# Autodesk Inventor assembly: 5A.00.03.01-IB-VTP-Rudder-Master-Assy
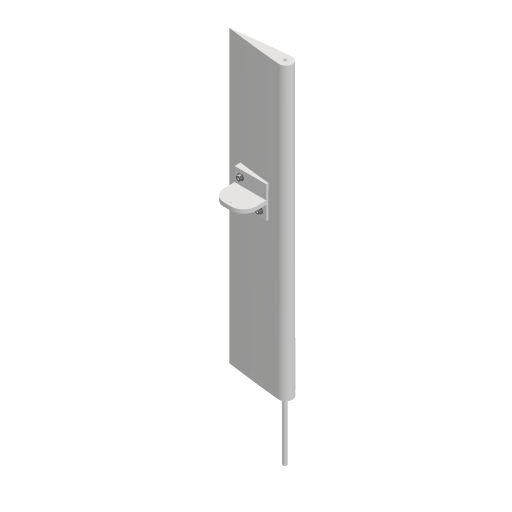
[picture p0: Inventor's stored thumbnail of the model, 512x512]
Saved by Autodesk Inventor 2024.3 (Build 283343000, 343)
## iProperties
Created: 2025-01-15
Part Number: 5A.00.03.01-IB-VTP-Rudder-Master-Assy
Document SubType Name: Assembly
Designer: inigo
Author: inigo
## Documents named in this file (11)
- C:\Users\inigo\OneDrive - University of Bristol\General - grp-Company A - AVDASI2 2024-25\CAD Files\Fuselage\VTP\5A.00.03.01-IB-VTP-Rudder-Master-Assy.iam
- C:\Users\inigo\OneDrive - University of Bristol\General - grp-Company A - AVDASI2 2024-25\CAD Files\Fuselage\VTP\5P.00.04.01-IB-VTP-Rudder-Right.ipt
- C:\Users\inigo\OneDrive - University of Bristol\General - grp-Company A - AVDASI2 2024-25\CAD Files\Fuselage\VTP\5P.00.05.01-IB-VTP-Rudder-Left.ipt
- C:\Users\inigo\OneDrive - University of Bristol\General - grp-Company A - AVDASI2 2024-25\CAD Files\Fuselage\VTP\5P.00.07.01-IB-VTP-Rudder-Bottom-Rib.ipt
- C:\Users\inigo\OneDrive - University of Bristol\General - grp-Company A - AVDASI2 2024-25\CAD Files\Fuselage\VTP\5P.00.08.01-IB-Rear-Spar.ipt
- C:\Users\inigo\OneDrive - University of Bristol\General - grp-Company A - AVDASI2 2024-25\CAD Files\Fuselage\VTP\5P.00.17.01-IB-VTP-Control-Horn.ipt
- C:\Users\inigo\OneDrive - University of Bristol\General - grp-Company A - AVDASI2 2024-25\CAD Files\Fuselage\VTP\5P.00.18.01-IB-VTP-Rudder-Top-Rib.ipt
- C:\Users\inigo\OneDrive - University of Bristol\General - grp-Company A - AVDASI2 2024-25\CAD Files\Fuselage\VTP\5P.00.21.01-IB-VTP-Rudder-Backplate.ipt
- C:\Users\inigo\Documents\Inventor\Content Center Files\R2024\en-US\ISO 4762(2)\ISO 4762 - M2 x 16ISO.ipt
- C:\Users\inigo\Documents\Inventor\Content Center Files\R2024\en-US\ISO 7089\ISO 7089 - 2 - 140 HV(1).ipt
- C:\Users\inigo\Documents\Inventor\Content Center Files\R2024\en-US\ISO 4032(2)\ISO 4032 - M2 - ISO.ipt
## Components (15 placed, 10 different names)
1. 5P.00.04.01-IB-VTP-Rudder-Right:1 — Mate:4, Mate:5, Flush:1, Mate:8, Mate:9, Mate:10, Mate:11, Mate:12, Flush:3
2. 5P.00.05.01-IB-VTP-Rudder-Left:1 — Mate:1, Mate:3, Mate:5, Flush:1, Mate:7, Mate:13, Mate:14
3. 5P.00.07.01-IB-VTP-Rudder-Bottom-Rib:1 — Mate:2, Mate:3, Mate:9
4. 5P.00.08.01-IB-Rear-Spar:1 — Mate:1, Mate:2, Mate:4, Mate:6, Flush:2
5. 5P.00.17.01-IB-VTP-Control-Horn:1 — Mate:10, Mate:11, Mate:12, Mate:17, Mate:20, Mate:21, Mate:22
6. 5P.00.18.01-IB-VTP-Rudder-Top-Rib:1 — Mate:6, Mate:7, Mate:8, Flush:2
7. 5P.00.21.01-IB-VTP-Rudder-Backplate:1 — Mate:13, Mate:14, Flush:3, Mate:24, Mate:26
8. ISO 4762 M2 x 16:1 — Mate:15, Mate:16, Mate:17, Mate:23, Mate:27
9. ISO 7089 2:1 — Mate:15, Mate:16, Mate:20
10. ISO 7089 2:2 — Mate:23, Mate:24, Mate:28
11. ISO 4762 M2 x 16:2 — Mate:21, Mate:25, Mate:29
12. ISO 7089 2:3 — Mate:22
13. ISO 7089 2:4 — Mate:25, Mate:26, Mate:30
14. ISO 4032 M2:1 — Mate:27, Mate:28
15. ISO 4032 M2:2 — Mate:29, Mate:30
## Relationships (33: Mate 30, Flush 3)
- Mate:1: 5P.00.05.01-IB-VTP-Rudder-Left:1 ↔ 5P.00.08.01-IB-Rear-Spar:1
- Mate:2: 5P.00.07.01-IB-VTP-Rudder-Bottom-Rib:1 ↔ 5P.00.08.01-IB-Rear-Spar:1
- Mate:3: 5P.00.05.01-IB-VTP-Rudder-Left:1 ↔ 5P.00.07.01-IB-VTP-Rudder-Bottom-Rib:1
- Mate:4: 5P.00.04.01-IB-VTP-Rudder-Right:1 ↔ 5P.00.08.01-IB-Rear-Spar:1
- Mate:5: 5P.00.04.01-IB-VTP-Rudder-Right:1 ↔ 5P.00.05.01-IB-VTP-Rudder-Left:1
- Flush:1: 5P.00.04.01-IB-VTP-Rudder-Right:1 ↔ 5P.00.05.01-IB-VTP-Rudder-Left:1
- Mate:6: 5P.00.08.01-IB-Rear-Spar:1 ↔ 5P.00.18.01-IB-VTP-Rudder-Top-Rib:1
- Mate:7: 5P.00.05.01-IB-VTP-Rudder-Left:1 ↔ 5P.00.18.01-IB-VTP-Rudder-Top-Rib:1
- Mate:8: 5P.00.04.01-IB-VTP-Rudder-Right:1 ↔ 5P.00.18.01-IB-VTP-Rudder-Top-Rib:1
- Mate:9: 5P.00.04.01-IB-VTP-Rudder-Right:1 ↔ 5P.00.07.01-IB-VTP-Rudder-Bottom-Rib:1
- Flush:2: 5P.00.08.01-IB-Rear-Spar:1 ↔ 5P.00.18.01-IB-VTP-Rudder-Top-Rib:1
- Mate:10: 5P.00.04.01-IB-VTP-Rudder-Right:1 ↔ 5P.00.17.01-IB-VTP-Control-Horn:1
- Mate:11 (-6 mm): 5P.00.04.01-IB-VTP-Rudder-Right:1 ↔ 5P.00.17.01-IB-VTP-Control-Horn:1
- Mate:12: 5P.00.04.01-IB-VTP-Rudder-Right:1 ↔ 5P.00.17.01-IB-VTP-Control-Horn:1
- Mate:13: 5P.00.05.01-IB-VTP-Rudder-Left:1 ↔ 5P.00.21.01-IB-VTP-Rudder-Backplate:1
- Mate:14: 5P.00.05.01-IB-VTP-Rudder-Left:1 ↔ 5P.00.21.01-IB-VTP-Rudder-Backplate:1
- Flush:3 (-6 mm): 5P.00.04.01-IB-VTP-Rudder-Right:1 ↔ 5P.00.21.01-IB-VTP-Rudder-Backplate:1
- Mate:15: ISO 4762 M2 x 16:1 ↔ ISO 7089 2:1
- Mate:16: ISO 4762 M2 x 16:1 ↔ ISO 7089 2:1
- Mate:17: 5P.00.17.01-IB-VTP-Control-Horn:1 ↔ ISO 4762 M2 x 16:1
- [Mate]: ISO 4762 M2 x 16:2 ↔ ISO 7089 2:3
- [Mate]: ISO 4762 M2 x 16:2 ↔ ISO 7089 2:3
- Mate:20: 5P.00.17.01-IB-VTP-Control-Horn:1 ↔ ISO 7089 2:1
- Mate:21: 5P.00.17.01-IB-VTP-Control-Horn:1 ↔ ISO 4762 M2 x 16:2
- Mate:22: 5P.00.17.01-IB-VTP-Control-Horn:1 ↔ ISO 7089 2:3
- Mate:23: ISO 4762 M2 x 16:1 ↔ ISO 7089 2:2
- Mate:24: 5P.00.21.01-IB-VTP-Rudder-Backplate:1 ↔ ISO 7089 2:2
- Mate:25: ISO 4762 M2 x 16:2 ↔ ISO 7089 2:4
- Mate:26: 5P.00.21.01-IB-VTP-Rudder-Backplate:1 ↔ ISO 7089 2:4
- Mate:27: ISO 4762 M2 x 16:1 ↔ ISO 4032 M2:1
- Mate:28: ISO 7089 2:2 ↔ ISO 4032 M2:1
- Mate:29: ISO 4762 M2 x 16:2 ↔ ISO 4032 M2:2
- Mate:30: ISO 7089 2:4 ↔ ISO 4032 M2:2
## Named parameters: d20_d17 = 0 mm, d21_d18 = 0 mm
